# Autodesk Inventor assembly: new_u64_2
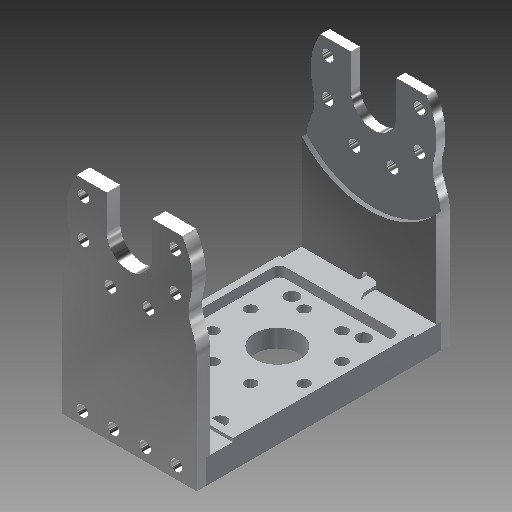
[picture p0: Inventor's stored thumbnail of the model, 512x512]
Saved by Autodesk Inventor 2018 (Build 220112000, 112)
## iProperties
Created: 2017-01-11
Part Number: new_u64_2
Document SubType Name: Assembly
Designer: steve
Mass: 24.0837 g
Surface Area: 102.457 cm^2
Volume: 12.1697 cm^3
Density: 1.97899 g/cm^3
Author: steve
## Documents named in this file (4)
- C:\Users\etd\Dropbox\SigmaBan\SigmaBanV2.1\new_U\new_u64_2.iam
- C:\Users\etd\Dropbox\SigmaBan\SigmaBanV2.1\new_U\new_base_u64.ipt
- C:\Users\etd\Dropbox\SigmaBan\SigmaBanV2.1\test_side_u64.ipt
- C:\Users\etd\Dropbox\SigmaBan\SigmaBanV2.1\test_side_u64_with_trace.ipt
## Components (3 placed, 3 different names)
1. new_base_u64:1 — Mate:6, Mate:7, Mate:8, Mate:9, Mate:10, Mate:11
2. test_side_u64:1 — Mate:6, Mate:10, Mate:11
3. test_side_u64_with_trace:1 — Mate:7, Mate:8, Mate:9
## Relationships (6: Mate 6)
- Mate:6: new_base_u64:1 ↔ test_side_u64:1
- Mate:7: new_base_u64:1 ↔ test_side_u64_with_trace:1
- Mate:8: new_base_u64:1 ↔ test_side_u64_with_trace:1
- Mate:9: new_base_u64:1 ↔ test_side_u64_with_trace:1
- Mate:10: new_base_u64:1 ↔ test_side_u64:1
- Mate:11: new_base_u64:1 ↔ test_side_u64:1
